# Autodesk Inventor assembly: TurnTable_140
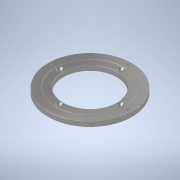
[picture p0: Inventor's stored thumbnail of the model, 180x180]
Saved by Autodesk Inventor 2024.3 (Build 283343010, 343A)
## iProperties
Created: 2021-11-29
Part Number: TurnTable_140
Document SubType Name: Assembly
Designer: satot
Mass: 567.745 g
Surface Area: 300.657 cm^2
Volume: 73.4469 cm^3
Density: 7.73 g/cm^3
Author: satot
## Documents named in this file (3)
- C:\Users\kshau\Documents\inventor\Create_ViperX\BasicParts\TurnTable\TurnTable_140\TurnTable_140.iam
- C:\Users\kshau\Documents\inventor\Create_ViperX\BasicParts\TurnTable\TurnTable_140\TurnTable140_Inner.ipt
- C:\Users\kshau\Documents\inventor\Create_ViperX\BasicParts\TurnTable\TurnTable_140\TurnTable_140_Outer.ipt
## Components (2 placed, 2 different names)
1. TurnTable140_Inner:1 — 回転:1
2. TurnTable_140_Outer:1 — 回転:1
## Relationships (1: RevoluteJoint 1)
- 回転:1 [RevoluteJoint]: TurnTable140_Inner:1 ↔ TurnTable_140_Outer:1
